# Autodesk Inventor assembly: F and B arm assembly
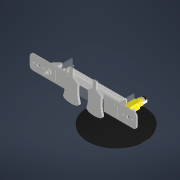
[picture p0: Inventor's stored thumbnail of the model, 180x180]
Saved by Autodesk Inventor 2021 (Build 250183000, 183)
## iProperties
Created: 2022-05-21
Part Number: F and B arm assembly
Document SubType Name: Assembly
Designer: techv
Author: techv
## Documents named in this file (11)
- D:\Projects\P_Baker Bot\Design\F and B assembly\F and B arm assembly.iam
- D:\Projects\P_Baker Bot\Design\dough arm assembly\poly carbonate plate.ipt
- D:\Projects\P_Baker Bot\Design\dough arm assembly\arm1.ipt
- D:\Projects\P_Baker Bot\Design\dough arm assembly\Roller.ipt
- D:\Projects\P_Baker Bot\Design\F and B assembly\arm2.ipt
- D:\Projects\A_Electronics CAD model\BO DC Motor.ipt
- D:\Projects\P_Baker Bot\Design\F and B assembly\l bracket.ipt
- D:\Projects\P_Baker Bot\Design\F and B assembly\3d mount for linear bearing.ipt
- D:\Projects\P_Baker Bot\Design\F and B assembly\3d mount for linear bearing and leadscrew.ipt
- D:\Projects\P_Baker Bot\Design\F and B assembly\Linear_rod_nut_8mm.ipt
- D:\Projects\P_Baker Bot\Design\F and B assembly\spatula.ipt
## Components (13 placed, 10 different names)
1. poly carbonate plate:1 — Mate:22
2. Roller:1 — Mate:1, Flush:1, Mate:5, Flush:9, Mate:7, Mate:8, Mate:9, Mate:15
3. arm1:1 — Flush:5, Flush:6, Flush:7, Flush:8, Mate:11, Mate:13, Flush:11, Mate:14, Flush:12, Mate:16, Mate:20, Mate:21
4. arm2:1 — Flush:5, Flush:6, Flush:9, Mate:12, Mate:14, Mate:15, Mate:17
5. arm2:2 — Mate:5, Flush:7, Flush:8, Mate:10
6. BO DC Motor:1 — Mate:7, Mate:8, Mate:9, Mate:22
7. l bracket:2 — Mate:10, Mate:11, Flush:10
8. l bracket:3 — Mate:12, Mate:13, Flush:10, Flush:11
9. 3d mount for linear bearing:1 — Angle:1
10. 3d mount for linear bearing and leadscrew:1 — Flush:12, Mate:16, Mate:17, Mate:18, Mate:19
11. Linear_rod_nut_8mm:1 — Mate:18, Mate:19
12. spatula:1 — Mate:20, Angle:1, Mate:21
13. spatula:2
## Relationships (28: Mate 18, Flush 9, Angle 1)
- Mate:1: Roller:1
- Flush:1: Roller:1
- Mate:5: Roller:1 ↔ arm2:2
- Flush:5: arm1:1 ↔ arm2:1
- Flush:6: arm1:1 ↔ arm2:1
- Flush:7: arm1:1 ↔ arm2:2
- Flush:8: arm1:1 ↔ arm2:2
- Flush:9 (3.641 mm): Roller:1 ↔ arm2:1
- Mate:7: Roller:1 ↔ BO DC Motor:1
- Mate:8: Roller:1 ↔ BO DC Motor:1
- Mate:9: Roller:1 ↔ BO DC Motor:1
- Mate:10: arm2:2 ↔ l bracket:2
- Mate:11: arm1:1 ↔ l bracket:2
- Mate:12: arm2:1 ↔ l bracket:3
- Mate:13: arm1:1 ↔ l bracket:3
- Flush:10: l bracket:2 ↔ l bracket:3
- Flush:11 (-15 mm): arm1:1 ↔ l bracket:3
- Mate:14: arm1:1 ↔ arm2:1
- Mate:15: Roller:1 ↔ arm2:1
- Flush:12: arm1:1 ↔ 3d mount for linear bearing and leadscrew:1
- Mate:16: arm1:1 ↔ 3d mount for linear bearing and leadscrew:1
- Mate:17: arm2:1 ↔ 3d mount for linear bearing and leadscrew:1
- Mate:18: 3d mount for linear bearing and leadscrew:1 ↔ Linear_rod_nut_8mm:1
- Mate:19: 3d mount for linear bearing and leadscrew:1 ↔ Linear_rod_nut_8mm:1
- Mate:20: arm1:1 ↔ spatula:1
- Angle:1 (0 deg): 3d mount for linear bearing:1 ↔ spatula:1
- Mate:21: arm1:1 ↔ spatula:1
- Mate:22 (60 mm): poly carbonate plate:1 ↔ BO DC Motor:1
